# Autodesk Inventor assembly: whole_case
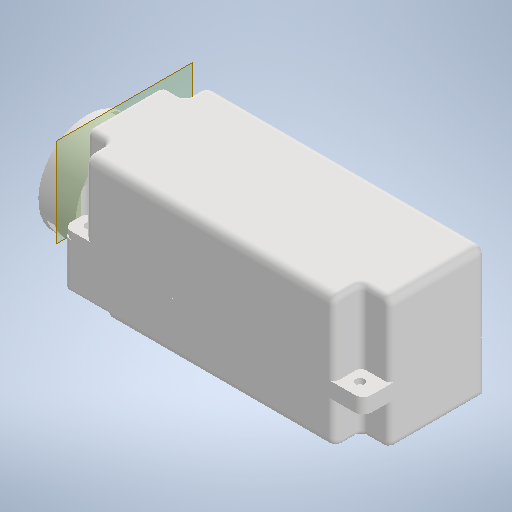
[picture p0: Inventor's stored thumbnail of the model, 512x512]
Saved by Autodesk Inventor 2025.2 (Build 292293000, 293)
## iProperties
Created: 2025-03-27
Part Number: whole_case
Document SubType Name: Assembly
Designer: Acer
Author: Acer
## Documents named in this file (3)
- C:\Users\Acer\Desktop\Projekty_Git\capacitor_teaser\3D_models\whole_case.iam
- C:\Users\Acer\Desktop\Projekty_Git\capacitor_teaser\3D_models\case_bottom.ipt
- C:\Users\Acer\Desktop\Projekty_Git\capacitor_teaser\3D_models\case_top.ipt
## Components (2 placed, 2 different names)
1. case_bottom:1 — Mate:1, Mate:2, Flush:1
2. case_top:1 — Mate:1, Mate:2, Flush:1
## Relationships (3: Mate 2, Flush 1)
- Mate:1: case_bottom:1 ↔ case_top:1
- Mate:2: case_bottom:1 ↔ case_top:1
- Flush:1: case_bottom:1 ↔ case_top:1
